# Autodesk Inventor assembly: Shooter Curve Assembly
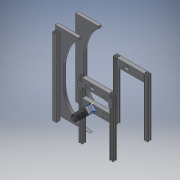
[picture p0: Inventor's stored thumbnail of the model, 180x180]
Saved by Autodesk Inventor 2018 (Build 220112000, 112)
## iProperties
Created: 2020-02-01
Part Number: Shooter Curve Assembly
Document SubType Name: Assembly
Designer: Weeb No1
Author: Weeb No1
## Documents named in this file (8)
- C:\Users\T3500STATIC\Documents\GitHub\2020CAD\Gabriel Inventor Files (Shooter, Drivebase)\Shooter Curve Assembly\Main Assembly File\Shooter Curve Assembly.iam
- C:\Users\T3500STATIC\Documents\GitHub\2020CAD\Gabriel Inventor Files (Shooter, Drivebase)\Shooter Curve Assembly\Part Files\Shooter Main Curve.ipt
- C:\Users\T3500STATIC\Documents\GitHub\2020CAD\Gabriel Inventor Files (Shooter, Drivebase)\Shooter Curve Assembly\Part Files\8020 1010 x 15.ipt
- C:\Users\T3500STATIC\Documents\GitHub\2020CAD\Gabriel Inventor Files (Shooter, Drivebase)\Shooter Curve Assembly\Part Files\1x2 5 in Beam Flywheel Mount.ipt
- C:\Users\T3500STATIC\Documents\GitHub\2020CAD\Over bumper intake\Parts\VersaPlanetary_v2_Single_Stage_10_1_with_775_Series.iam
- C:\Users\T3500STATIC\Documents\GitHub\2020CAD\Gabriel Inventor Files (Shooter, Drivebase)\Shooter Curve Assembly\Part Files\1x2 7 in Beam Motor Mount.ipt
- C:\Users\T3500STATIC\Documents\GitHub\2020CAD\Gabriel Inventor Files (Shooter, Drivebase)\Gussets\L-Gusset 3 Hole 0.25in Hole.ipt
- C:\Users\T3500STATIC\Documents\GitHub\2020CAD\Gabriel Inventor Files (Shooter, Drivebase)\Shooter Curve Assembly\Part Files\1x1 20 in Curve Support Beam.ipt
## Components (16 placed, 7 different names)
1. Shooter Main Curve:1 — Flush:1, Mate:1, Mate:2, Flush:2, Flush:3, Flush:18, Flush:20, Mate:68, Flush:36, Flush:37
2. 8020 1010 x 15:1 — Flush:1, Mate:1, Flush:5, Flush:6, Mate:7, Flush:11, Flush:14, Flush:18, Flush:23, Flush:24, Mate:51, Mate:56, Mate:60
3. 8020 1010 x 15:2 — Flush:4, Mate:3, Flush:7, Mate:9, Flush:15, Flush:19, Flush:22, Flush:25
4. Shooter Main Curve:2 — Mate:2, Flush:2, Flush:3, Flush:4, Mate:3, Flush:19, Flush:21, Mate:67, Flush:35, Flush:38
5. 8020 1010 x 15:3 — Flush:5, Flush:6, Flush:10, Flush:12, Flush:13, Flush:20, Mate:11, Flush:23, Mate:50, Flush:34, Mate:63, Mate:65
6. 8020 1010 x 15:4 — Flush:7, Flush:10, Flush:17, Flush:21, Mate:10, Flush:22
7. 1x2 5 in Beam Flywheel Mount:1 — Mate:9, Flush:15, Flush:17, Mate:10, Flush:25
8. 1x2 5 in Beam Flywheel Mount:2 — Mate:7, Flush:11, Flush:12, Flush:13, Flush:14, Mate:11, Flush:24, Mate:55, Mate:57, Mate:58, Mate:59, Mate:61, Mate:62, Mate:64, Mate:66
9. VersaPlanetary_v2_Single_Stage_10_1_with_775_Series:1 [sub-assembly] — Mate:52, Mate:53, Mate:54
10. 1x2 7 in Beam Motor Mount:1 — Mate:50, Mate:51, Flush:34, Mate:52, Mate:53, Mate:54
11. L-Gusset 3 Hole 0.25in Hole:1 — Mate:61, Mate:62, Mate:63
12. L-Gusset 3 Hole 0.25in Hole:2 — Mate:55, Mate:56, Mate:57
13. L-Gusset 3 Hole 0.25in Hole:3 — Mate:58, Mate:59, Mate:60
14. L-Gusset 3 Hole 0.25in Hole:4 — Mate:64, Mate:65, Mate:66
15. 1x1 20 in Curve Support Beam:1 — Mate:68, Flush:36, Flush:37
16. 1x1 20 in Curve Support Beam:2 — Mate:67, Flush:35, Flush:38
## Relationships (53: Flush 27, Mate 26)
- Flush:1 (203.2 mm): Shooter Main Curve:1 ↔ 8020 1010 x 15:1
- Mate:1 (25.4 mm): Shooter Main Curve:1 ↔ 8020 1010 x 15:1
- Mate:2 (114.3 mm): Shooter Main Curve:1 ↔ Shooter Main Curve:2
- Flush:2: Shooter Main Curve:1 ↔ Shooter Main Curve:2
- Flush:3: Shooter Main Curve:1 ↔ Shooter Main Curve:2
- Flush:4 (203.2 mm): 8020 1010 x 15:2 ↔ Shooter Main Curve:2
- Mate:3 (25.4 mm): 8020 1010 x 15:2 ↔ Shooter Main Curve:2
- Flush:5: 8020 1010 x 15:1 ↔ 8020 1010 x 15:3
- Flush:6: 8020 1010 x 15:1 ↔ 8020 1010 x 15:3
- Flush:7: 8020 1010 x 15:2 ↔ 8020 1010 x 15:4
- Flush:10: 8020 1010 x 15:3 ↔ 8020 1010 x 15:4
- Mate:7: 8020 1010 x 15:1 ↔ 1x2 5 in Beam Flywheel Mount:2
- Flush:11: 8020 1010 x 15:1 ↔ 1x2 5 in Beam Flywheel Mount:2
- Flush:12: 8020 1010 x 15:3 ↔ 1x2 5 in Beam Flywheel Mount:2
- Flush:13: 8020 1010 x 15:3 ↔ 1x2 5 in Beam Flywheel Mount:2
- Flush:14: 8020 1010 x 15:1 ↔ 1x2 5 in Beam Flywheel Mount:2
- Mate:9: 8020 1010 x 15:2 ↔ 1x2 5 in Beam Flywheel Mount:1
- Flush:15: 8020 1010 x 15:2 ↔ 1x2 5 in Beam Flywheel Mount:1
- Flush:17: 8020 1010 x 15:4 ↔ 1x2 5 in Beam Flywheel Mount:1
- Flush:18 (-37.846 mm): Shooter Main Curve:1 ↔ 8020 1010 x 15:1
- Flush:19 (-37.846 mm): 8020 1010 x 15:2 ↔ Shooter Main Curve:2
- Flush:20 (-37.846 mm): Shooter Main Curve:1 ↔ 8020 1010 x 15:3
- Flush:21 (-37.846 mm): Shooter Main Curve:2 ↔ 8020 1010 x 15:4
- Mate:10: 8020 1010 x 15:4 ↔ 1x2 5 in Beam Flywheel Mount:1
- Mate:11: 8020 1010 x 15:3 ↔ 1x2 5 in Beam Flywheel Mount:2
- Flush:22: 8020 1010 x 15:2 ↔ 8020 1010 x 15:4
- Flush:23: 8020 1010 x 15:1 ↔ 8020 1010 x 15:3
- Flush:24: 8020 1010 x 15:1 ↔ 1x2 5 in Beam Flywheel Mount:2
- Flush:25: 8020 1010 x 15:2 ↔ 1x2 5 in Beam Flywheel Mount:1
- Mate:50: 8020 1010 x 15:3 ↔ 1x2 7 in Beam Motor Mount:1
- Mate:51: 8020 1010 x 15:1 ↔ 1x2 7 in Beam Motor Mount:1
- Flush:34: 8020 1010 x 15:3 ↔ 1x2 7 in Beam Motor Mount:1
- Mate:52: VersaPlanetary_v2_Single_Stage_10_1_with_775_Series:1 ↔ 1x2 7 in Beam Motor Mount:1
- Mate:53: VersaPlanetary_v2_Single_Stage_10_1_with_775_Series:1 ↔ 1x2 7 in Beam Motor Mount:1
- Mate:54: VersaPlanetary_v2_Single_Stage_10_1_with_775_Series:1 ↔ 1x2 7 in Beam Motor Mount:1
- Mate:55: 1x2 5 in Beam Flywheel Mount:2 ↔ L-Gusset 3 Hole 0.25in Hole:2
- Mate:56: 8020 1010 x 15:1 ↔ L-Gusset 3 Hole 0.25in Hole:2
- Mate:57: 1x2 5 in Beam Flywheel Mount:2 ↔ L-Gusset 3 Hole 0.25in Hole:2
- Mate:58: 1x2 5 in Beam Flywheel Mount:2 ↔ L-Gusset 3 Hole 0.25in Hole:3
- Mate:59: 1x2 5 in Beam Flywheel Mount:2 ↔ L-Gusset 3 Hole 0.25in Hole:3
- Mate:60: 8020 1010 x 15:1 ↔ L-Gusset 3 Hole 0.25in Hole:3
- Mate:61: 1x2 5 in Beam Flywheel Mount:2 ↔ L-Gusset 3 Hole 0.25in Hole:1
- Mate:62: 1x2 5 in Beam Flywheel Mount:2 ↔ L-Gusset 3 Hole 0.25in Hole:1
- Mate:63: 8020 1010 x 15:3 ↔ L-Gusset 3 Hole 0.25in Hole:1
- Mate:64: 1x2 5 in Beam Flywheel Mount:2 ↔ L-Gusset 3 Hole 0.25in Hole:4
- Mate:65: 8020 1010 x 15:3 ↔ L-Gusset 3 Hole 0.25in Hole:4
- Mate:66: 1x2 5 in Beam Flywheel Mount:2 ↔ L-Gusset 3 Hole 0.25in Hole:4
- Mate:67: Shooter Main Curve:2 ↔ 1x1 20 in Curve Support Beam:2
- Flush:35 (-25.4 mm): Shooter Main Curve:2 ↔ 1x1 20 in Curve Support Beam:2
- Mate:68: Shooter Main Curve:1 ↔ 1x1 20 in Curve Support Beam:1
- Flush:36 (-25.4 mm): Shooter Main Curve:1 ↔ 1x1 20 in Curve Support Beam:1
- Flush:37 (6.35 mm): Shooter Main Curve:1 ↔ 1x1 20 in Curve Support Beam:1
- Flush:38 (6.35 mm): Shooter Main Curve:2 ↔ 1x1 20 in Curve Support Beam:2
